# Autodesk Inventor assembly: Toolhead
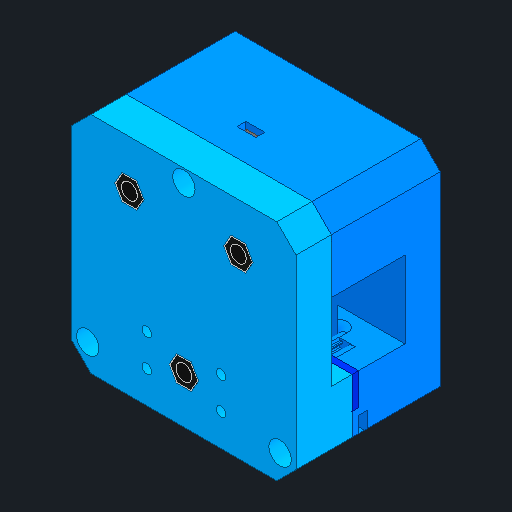
[picture p0: Inventor's stored thumbnail of the model, 512x512]
Saved by Autodesk Inventor 2025.1 (Build 291241000, 241)
## iProperties
Created: 2024-10-17
Part Number: Toolhead
Document SubType Name: Assembly
Designer: jerem
Author: jerem
## Documents named in this file (10)
- C:\Users\jerem\Documents\GitHub\Perovskite-Automated-Synthesis-System\CAD\Toolhead\Toolhead.iam
- C:\Users\jerem\Documents\GitHub\Perovskite-Automated-Synthesis-System\CAD\Non 3D Printed Parts\Printer Wheel.ipt
- C:\Users\jerem\Documents\GitHub\Perovskite-Automated-Synthesis-System\CAD\Toolhead\Toolhead Base.ipt
- C:\Users\jerem\Documents\GitHub\Perovskite-Automated-Synthesis-System\CAD\Toolhead\Toolhead Cover.ipt
- C:\Users\jerem\Documents\GitHub\Perovskite-Automated-Synthesis-System\CAD\Toolhead\Belt Holders.ipt
- C:\Users\jerem\Documents\GitHub\Perovskite-Automated-Synthesis-System\CAD\Non 3D Printed Parts\Screws\M3x16.ipt
- C:\Users\jerem\Documents\GitHub\Perovskite-Automated-Synthesis-System\CAD\Non 3D Printed Parts\Nuts\M3 Square Nut.ipt
- C:\Users\jerem\Documents\GitHub\Perovskite-Automated-Synthesis-System\CAD\Non 3D Printed Parts\Screws\M5x40.ipt
- C:\Users\jerem\Documents\GitHub\Perovskite-Automated-Synthesis-System\CAD\Non 3D Printed Parts\Nuts\M5 Nut.ipt
- C:\Users\jerem\Documents\GitHub\Perovskite-Automated-Synthesis-System\CAD\Non 3D Printed Parts\Screws\M3x12.ipt
## Components (27 placed, 9 different names)
1. Printer Wheel:1 — Mate:2, Mate:5, Mate:10, Mate:38
2. Printer Wheel:2 — Mate:3, Mate:6, Mate:40
3. Printer Wheel:3 — Mate:1, Mate:4, Mate:9, Mate:39
4. Toolhead Base:1 — Mate:1, Mate:2, Mate:3, Mate:4, Mate:5, Mate:6, Mate:12, Mate:13, Mate:14, Mate:15, Flush:2, Flush:3, Mate:16, Mate:26, Mate:27, Mate:28, Mate:29, Mate:30, Mate:31, Mate:33, Angle:4, Mate:34, Angle:5, Angle:6, Angle:7, Mate:41, Mate:42, Angle:43, Mate:43, Angle:47, Mate:51, Mate:52
5. Toolhead Cover:1 — Mate:9, Mate:10, Mate:18, Mate:19, Mate:20, Mate:21, Angle:1, Angle:2, Angle:3, Mate:22, Mate:23, Mate:24, Mate:25, Mate:32, Angle:42, Mate:41, Mate:44, Angle:44, Angle:45, Angle:46, Flush:46, Flush:47, Flush:48, Mate:48, Mate:49, Mate:50, Mate:53, Mate:54, Mate:55, Mate:56, Mate:57
6. Belt Holders:1 — Mate:12, Mate:15, Flush:2, Mate:17
7. Belt Holders:2 — Mate:13, Mate:14, Flush:3
8. M3x16:1 — Mate:16, Mate:17
9. M3 Square Nut:1 — Mate:19, Angle:3, Mate:22
10. M3 Square Nut:2 — Mate:21, Mate:23, Angle:42
11. M3 Square Nut:3 — Mate:18, Angle:1, Mate:24
12. M3 Square Nut:4 — Mate:20, Angle:2, Mate:25
13. M5x40:1 — Mate:26, Mate:27, Mate:37
14. M5x40:2 — Mate:28, Mate:29, Mate:36
15. M5x40:3 — Mate:30, Mate:31, Mate:35
16. M3x12:1 — Mate:32, Mate:44
17. M3 Square Nut:5 — Mate:33, Angle:4, Mate:34
18. M5 Nut:1 — Mate:35, Mate:40, Angle:5
19. M5 Nut:2 — Mate:37, Mate:39, Angle:7
20. M5 Nut:3 — Mate:36, Mate:38, Angle:6
21. M3 Square Nut:6 — Mate:42, Angle:43, Mate:43
22. M5 Nut:4 — Angle:44, Flush:48, Mate:48
23. M5 Nut:5 — Angle:45, Flush:47, Mate:49
24. M5 Nut:6 — Angle:46, Flush:46, Mate:50
25. M3 Square Nut:7 — Angle:47, Mate:51, Mate:52
26. M3x12:2 — Mate:53, Mate:54
27. M3x12:3 — Mate:55, Mate:56
## Relationships (69: Mate 51, Angle 13, Flush 5)
- Mate:1: Printer Wheel:3 ↔ Toolhead Base:1
- Mate:2: Printer Wheel:1 ↔ Toolhead Base:1
- Mate:3: Printer Wheel:2 ↔ Toolhead Base:1
- Mate:4: Printer Wheel:3 ↔ Toolhead Base:1
- Mate:5: Printer Wheel:1 ↔ Toolhead Base:1
- Mate:6: Printer Wheel:2 ↔ Toolhead Base:1
- Mate:9: Printer Wheel:3 ↔ Toolhead Cover:1
- Mate:10: Printer Wheel:1 ↔ Toolhead Cover:1
- Mate:12: Toolhead Base:1 ↔ Belt Holders:1
- Mate:13: Toolhead Base:1 ↔ Belt Holders:2
- Mate:14: Toolhead Base:1 ↔ Belt Holders:2
- Mate:15: Toolhead Base:1 ↔ Belt Holders:1
- Flush:2: Toolhead Base:1 ↔ Belt Holders:1
- Flush:3: Toolhead Base:1 ↔ Belt Holders:2
- Mate:16: Toolhead Base:1 ↔ M3x16:1
- Mate:17: Belt Holders:1 ↔ M3x16:1
- Mate:18: Toolhead Cover:1 ↔ M3 Square Nut:3
- Mate:19: Toolhead Cover:1 ↔ M3 Square Nut:1
- Mate:20: Toolhead Cover:1 ↔ M3 Square Nut:4
- Mate:21: Toolhead Cover:1 ↔ M3 Square Nut:2
- Angle:1 (0 deg): Toolhead Cover:1 ↔ M3 Square Nut:3
- Angle:2 (0 deg): Toolhead Cover:1 ↔ M3 Square Nut:4
- Angle:3 (0 deg): Toolhead Cover:1 ↔ M3 Square Nut:1
- Mate:22: Toolhead Cover:1 ↔ M3 Square Nut:1
- Mate:23: Toolhead Cover:1 ↔ M3 Square Nut:2
- Mate:24: Toolhead Cover:1 ↔ M3 Square Nut:3
- Mate:25: Toolhead Cover:1 ↔ M3 Square Nut:4
- Mate:26: Toolhead Base:1 ↔ M5x40:1
- Mate:27: Toolhead Base:1 ↔ M5x40:1
- Mate:28: Toolhead Base:1 ↔ M5x40:2
- Mate:29: Toolhead Base:1 ↔ M5x40:2
- Mate:30: Toolhead Base:1 ↔ M5x40:3
- Mate:31: Toolhead Base:1 ↔ M5x40:3
- Mate:32: Toolhead Cover:1 ↔ M3x12:1
- Mate:33: Toolhead Base:1 ↔ M3 Square Nut:5
- Angle:4 (0 deg): Toolhead Base:1 ↔ M3 Square Nut:5
- Mate:34: Toolhead Base:1 ↔ M3 Square Nut:5
- Mate:35: M5x40:3 ↔ M5 Nut:1
- Mate:36: M5x40:2 ↔ M5 Nut:3
- Mate:37: M5x40:1 ↔ M5 Nut:2
- Mate:38: Printer Wheel:1 ↔ M5 Nut:3
- Mate:39: Printer Wheel:3 ↔ M5 Nut:2
- Mate:40: Printer Wheel:2 ↔ M5 Nut:1
- Angle:42 (0 deg): Toolhead Cover:1 ↔ M3 Square Nut:2
- Angle:5 (0 deg): Toolhead Base:1 ↔ M5 Nut:1
- Angle:6 (0 deg): Toolhead Base:1 ↔ M5 Nut:3
- Angle:7 (0 deg): Toolhead Base:1 ↔ M5 Nut:2
- Mate:41: Toolhead Base:1 ↔ Toolhead Cover:1
- Mate:42: Toolhead Base:1 ↔ M3 Square Nut:6
- Angle:43 (0 deg): Toolhead Base:1 ↔ M3 Square Nut:6
- Mate:43: Toolhead Base:1 ↔ M3 Square Nut:6
- Mate:44: Toolhead Cover:1 ↔ M3x12:1
- Angle:44 (0 deg): Toolhead Cover:1 ↔ M5 Nut:4
- Angle:45 (0 deg): Toolhead Cover:1 ↔ M5 Nut:5
- Angle:46 (0 deg): Toolhead Cover:1 ↔ M5 Nut:6
- Flush:46: Toolhead Cover:1 ↔ M5 Nut:6
- Flush:47: Toolhead Cover:1 ↔ M5 Nut:5
- Flush:48: Toolhead Cover:1 ↔ M5 Nut:4
- Mate:48: Toolhead Cover:1 ↔ M5 Nut:4
- Mate:49: Toolhead Cover:1 ↔ M5 Nut:5
- Mate:50: Toolhead Cover:1 ↔ M5 Nut:6
- Angle:47 (0 deg): Toolhead Base:1 ↔ M3 Square Nut:7
- Mate:51: Toolhead Base:1 ↔ M3 Square Nut:7
- Mate:52: Toolhead Base:1 ↔ M3 Square Nut:7
- Mate:53: Toolhead Cover:1 ↔ M3x12:2
- Mate:54: Toolhead Cover:1 ↔ M3x12:2
- Mate:55: Toolhead Cover:1 ↔ M3x12:3
- Mate:56: Toolhead Cover:1 ↔ M3x12:3
- Mate:57: Toolhead Cover:1
